# Autodesk Inventor assembly: Drill Jig Assembly v2
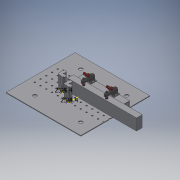
[picture p0: Inventor's stored thumbnail of the model, 180x180]
Saved by Autodesk Inventor 2018 (Build 220112000, 112)
## iProperties
Created: 2018-12-05
Part Number: Drill Jig Assembly v2
Document SubType Name: Assembly
Designer: gbgic
Author: gbgic
## Documents named in this file (6)
- C:\Users\Gabriel\Documents\GitHub\2019CAD\Drill Jig Files\Drill Jig Assembly v2.iam
- C:\Users\Gabriel\Documents\GitHub\2019CAD\Drill Jig Files\Drill Jig Base.ipt
- C:\Users\Gabriel\Documents\GitHub\2019CAD\Drill Jig Files\Toggle Clamp Files\305-U.iam
- C:\Users\Gabriel\Documents\GitHub\2019CAD\Drill Jig Files\Jig2.1_1x1_Bolt_Pattern_PIN.ipt
- C:\Users\Gabriel\Documents\GitHub\2019CAD\Drill Jig Files\Clamp Mount Aligner v2.ipt
- C:\Users\Gabriel\Documents\GitHub\2019CAD\Drill Jig Files\1x2 Beam Test.ipt
## Components (7 placed, 5 different names)
1. Drill Jig Base:1 — Mate:7, Mate:8, Mate:9, Mate:10, Mate:11, Mate:12
2. 305-U:1 [sub-assembly] — Mate:13
3. 305-U:2 [sub-assembly] — Mate:14
4. Jig2.1_1x1_Bolt_Pattern_PIN:1 — Mate:7, Mate:8
5. Jig2.1_1x1_Bolt_Pattern_PIN:2 — Mate:9, Mate:10
6. Clamp Mount Aligner v2:1 — Mate:11, Mate:12, Mate:13, Mate:14
7. 1x2 Beam Test:1
## Relationships (8: Mate 8)
- Mate:7: Drill Jig Base:1 ↔ Jig2.1_1x1_Bolt_Pattern_PIN:1
- Mate:8: Drill Jig Base:1 ↔ Jig2.1_1x1_Bolt_Pattern_PIN:1
- Mate:9: Drill Jig Base:1 ↔ Jig2.1_1x1_Bolt_Pattern_PIN:2
- Mate:10: Drill Jig Base:1 ↔ Jig2.1_1x1_Bolt_Pattern_PIN:2
- Mate:11: Drill Jig Base:1 ↔ Clamp Mount Aligner v2:1
- Mate:12: Drill Jig Base:1 ↔ Clamp Mount Aligner v2:1
- Mate:13: 305-U:1 ↔ Clamp Mount Aligner v2:1
- Mate:14: 305-U:2 ↔ Clamp Mount Aligner v2:1
